# Autodesk Inventor assembly: Rail_AssemblyV2_0
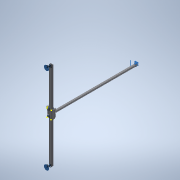
[picture p0: Inventor's stored thumbnail of the model, 180x180]
Saved by Autodesk Inventor 2021 (Build 250183000, 183)
## iProperties
Created: 2021-01-25
Part Number: Rail_AssemblyV2_0
Document SubType Name: Assembly
Designer: Jorian Brusind
Mass: 3786.54 g
Surface Area: 19508.5 cm^2
Volume: 2323.9 cm^3
Density: 1.62939 g/cm^3
Author: Jorian Brusind
## Documents named in this file (26)
- C:\Users\Jorian Bruslind\Documents\GitHub\PersonalProjects\HyperRail\Inventor Files\Rail_AssemblyV2_0.iam
- C:\Users\Jorian Bruslind\Documents\GitHub\PersonalProjects\Inventor Projects\Useful models\NEMA_Steppers\NEMA23\23HS8430B.ipt
- C:\Users\Jorian Bruslind\Documents\GitHub\PersonalProjects\HyperRail\Inventor Files\NEMA23_StepperonlineMount.ipt
- C:\Users\Jorian Bruslind\Documents\GitHub\PersonalProjects\Inventor Projects\Useful models\8020_Sets\IPT_20_Series\IPT_20_Series\20-2040_200mm.ipt
- C:\Users\Jorian Bruslind\Documents\GitHub\PersonalProjects\HyperRail\Inventor Files\2804S_NEMA2115_1Gearbox.ipt
- C:\Users\Jorian Bruslind\Documents\GitHub\PersonalProjects\HyperRail\Inventor Files\SmallBelt_LargePulley.ipt
- C:\Users\Jorian Bruslind\Documents\GitHub\PersonalProjects\HyperRail\PCB Files\Integrated Stepper Motor Driver\ExportSTEP\Main.iam
- C:\Users\Jorian Bruslind\Documents\GitHub\PersonalProjects\HyperRail\Inventor Files\NEMA23_Shroud.ipt
- C:\Users\Jorian Bruslind\Documents\GitHub\PersonalProjects\Inventor Projects\Useful models\8020_Sets\IPT_20_Series\IPT_20_Series\20-4040_2m.ipt
- C:\Users\Jorian Bruslind\Documents\GitHub\PersonalProjects\HyperRail\Inventor Files\98952A059_ALUM MALE-FEM THRDED HEX STANDOFF.ipt
- C:\Users\Jorian Bruslind\Documents\GitHub\PersonalProjects\HyperRail\Inventor Files\95783A039_NYLON 6-6 MALE-FEM THRDED HEX STANDOFF.ipt
- C:\Users\Jorian Bruslind\Documents\GitHub\PersonalProjects\HyperRail\Inventor Files\Integrated_Stepper_NEMA23_Mount.ipt
- C:\Users\Jorian Bruslind\Documents\GitHub\PersonalProjects\HyperRail\Inventor Files\Foot_Spacer.ipt
- C:\Users\Jorian Bruslind\Documents\GitHub\PersonalProjects\Inventor Projects\Useful models\Metric bolt\Bolt M5 50mm.ipt
- C:\Users\Jorian Bruslind\Documents\GitHub\PersonalProjects\Inventor Projects\Useful models\Metric nuts\Nut M5.ipt
- C:\Users\Jorian Bruslind\Documents\GitHub\PersonalProjects\HyperRail\Inventor Files\Bottom_Foot.ipt
- C:\Users\Jorian Bruslind\Documents\GitHub\PersonalProjects\HyperRail\Inventor Files\120deg_Tslot_Gusset.ipt
- C:\Users\Jorian Bruslind\Documents\GitHub\PersonalProjects\HyperRail\Inventor Files\90deg_4040Bracket.ipt
- C:\Users\Jorian Bruslind\Documents\GitHub\PersonalProjects\HyperRail\Inventor Files\X_Carriage_V2_0.iam
- C:\Users\Jorian Bruslind\Documents\GitHub\PersonalProjects\HyperRail\Inventor Files\11mm_BearingWheel.ipt
- C:\Users\Jorian Bruslind\Documents\GitHub\PersonalProjects\HyperRail\Inventor Files\X_CarriageR_V2_0.iam
- C:\Users\Jorian Bruslind\Documents\GitHub\PersonalProjects\Inventor Projects\Useful models\8020_Sets\IPT_40_Series\Extra_40_Series\HFS5-4060-4000\HFS5-4060-2125.ipt
- C:\Users\Jorian Bruslind\Documents\GitHub\PersonalProjects\Inventor Projects\Useful models\8020_Sets\IPT_20_Series\IPT_20_Series\20-2040_150mm.ipt
- C:\Users\Jorian Bruslind\Documents\GitHub\PersonalProjects\HyperRail\Inventor Files\RightAngle_Bracket_60mm.ipt
- C:\Users\Jorian Bruslind\Documents\GitHub\PersonalProjects\HyperRail\Inventor Files\X_CarriageR_V2_0_Short.iam
- C:\Users\Jorian Bruslind\Documents\GitHub\PersonalProjects\HyperRail\Inventor Files\X_CarriageL_V2_0_Short.iam
## Components (40 placed, 25 different names)
1. 23HS8430B:1 — Mate:127, Angle:3, Mate:158, Mate:177, Mate:179, Mate:180, Mate:181, Mate:182, Mate:183, Mate:184, Mate:185, Mate:264, Mate:265, Mate:295
2. NEMA23_StepperonlineMount:1 — Angle:2, Mate:98, Mate:128, Mate:255, Mate:258, Mate:259, Mate:289, Flush:99, Mate:290, Mate:303, Mate:304, Flush:107, Flush:108
3. 20-2040_200mm:1 — Mate:253, Flush:83, Flush:84, Flush:88, Mate:284, Mate:297, Mate:301, Mate:302, Flush:111, Flush:112
4. 2804S_NEMA2115_1Gearbox:1 — Angle:2, Mate:98, Mate:127, Mate:128, Angle:3, Mate:158, Mate:204, Flush:66, Flush:86
5. SmallBelt_LargePulley:1 — Mate:204, Flush:66
6. Main:1 [sub-assembly] — Mate:291, Mate:292, Mate:293
7. 20-4040_2m:2 — Mate:230, Flush:69, Flush:70, Mate:231, Flush:71, Flush:72, Mate:232, Flush:73, Mate:233, Mate:234, Flush:74, Mate:288, Flush:97, Flush:98
8. NEMA23_Shroud:1 — Mate:264, Mate:265, Flush:86, Mate:294
9. 98952A059_ALUM MALE-FEM THRDED HEX STANDOFF:1 — Mate:180, Mate:181, Mate:186, Mate:191
10. 98952A059_ALUM MALE-FEM THRDED HEX STANDOFF:2 — Mate:184, Mate:185, Mate:189, Mate:192
11. 98952A059_ALUM MALE-FEM THRDED HEX STANDOFF:3 — Mate:177, Mate:179, Mate:187, Mate:190
12. 98952A059_ALUM MALE-FEM THRDED HEX STANDOFF:4 — Mate:182, Mate:183, Mate:188, Mate:193
13. 95783A039_NYLON 6-6 MALE-FEM THRDED HEX STANDOFF:1 — Mate:188, Mate:193
14. 95783A039_NYLON 6-6 MALE-FEM THRDED HEX STANDOFF:2 — Mate:186, Mate:191
15. 95783A039_NYLON 6-6 MALE-FEM THRDED HEX STANDOFF:3 — Mate:187, Mate:190
16. 95783A039_NYLON 6-6 MALE-FEM THRDED HEX STANDOFF:4 — Mate:189, Mate:192
17. Bolt M5 50mm:1 — Mate:224, Mate:245, Mate:246, Mate:247, Mate:269
18. Nut M5:1 — Mate:226, Mate:247
19. Nut M5:2 — Mate:244, Flush:78, Mate:246
20. Bottom_Foot:1 — Mate:224, Mate:226, Mate:245, Flush:81, Flush:93
21. 120deg_Tslot_Gusset:1 — Mate:230, Flush:69, Flush:70
22. 120deg_Tslot_Gusset:2 — Mate:231, Flush:71, Flush:72
23. 90deg_4040Bracket:1 — Mate:232, Flush:73, Mate:233, Flush:75
24. 90deg_4040Bracket:2 — Mate:234, Flush:74, Flush:75
25. Foot_Spacer:1 — Mate:244, Flush:78, Mate:269, Mate:283, Flush:94
26. Foot_Spacer:2 — Mate:250, Mate:281, Flush:91, Flush:92, Mate:282
27. Bottom_Foot:2 — Mate:249, Mate:251, Flush:81, Flush:93
28. Bolt M5 50mm:2 — Mate:249, Mate:250, Mate:251, Mate:282
29. X_Carriage_V2_0:1 [sub-assembly] — Mate:253, Flush:83, Flush:84, Flush:109, Mate:309, Flush:113
30. 11mm_BearingWheel:1 — Mate:255, Mate:290
31. 11mm_BearingWheel:2 — Mate:258, Mate:259, Flush:109
32. 20-2040_200mm:2 — Flush:88, Mate:286, Flush:96, Mate:305, Flush:111, Mate:312, Flush:114
33. HFS5-4060-2125:1 — Mate:277, Mate:278, Mate:279, Mate:280, Mate:281, Flush:91, Flush:92, Mate:283, Flush:94, Mate:284, Flush:114
34. 20-2040_150mm:1 — Mate:286, Flush:96, Mate:288, Flush:97, Flush:98, Mate:289, Flush:99, Mate:310
35. Integrated_Stepper_NEMA23_Mount:1 — Mate:291, Mate:292, Mate:293, Mate:294, Mate:295
36. X_CarriageR_V2_0:2 [sub-assembly] — Mate:297, Mate:308, Flush:112, Flush:113, Mate:311
37. RightAngle_Bracket_60mm:1 — Mate:301, Mate:304, Flush:107
38. RightAngle_Bracket_60mm:2 — Mate:302, Mate:303, Flush:108
39. X_CarriageR_V2_0_Short:1 [sub-assembly] — Mate:305, Mate:308, Mate:309, Mate:310
40. X_CarriageL_V2_0_Short:1 [sub-assembly] — Mate:311, Mate:312
## Relationships (101: Mate 70, Flush 29, Angle 2)
- Angle:2 (0 deg): NEMA23_StepperonlineMount:1 ↔ 2804S_NEMA2115_1Gearbox:1
- Mate:98: NEMA23_StepperonlineMount:1 ↔ 2804S_NEMA2115_1Gearbox:1
- Mate:127: 23HS8430B:1 ↔ 2804S_NEMA2115_1Gearbox:1
- Mate:128: NEMA23_StepperonlineMount:1 ↔ 2804S_NEMA2115_1Gearbox:1
- Angle:3 (0 deg): 23HS8430B:1 ↔ 2804S_NEMA2115_1Gearbox:1
- Mate:158: 23HS8430B:1 ↔ 2804S_NEMA2115_1Gearbox:1
- Mate:177: 23HS8430B:1 ↔ 98952A059_ALUM MALE-FEM THRDED HEX STANDOFF:3
- Mate:179: 23HS8430B:1 ↔ 98952A059_ALUM MALE-FEM THRDED HEX STANDOFF:3
- Mate:180: 23HS8430B:1 ↔ 98952A059_ALUM MALE-FEM THRDED HEX STANDOFF:1
- Mate:181: 23HS8430B:1 ↔ 98952A059_ALUM MALE-FEM THRDED HEX STANDOFF:1
- Mate:182: 23HS8430B:1 ↔ 98952A059_ALUM MALE-FEM THRDED HEX STANDOFF:4
- Mate:183: 23HS8430B:1 ↔ 98952A059_ALUM MALE-FEM THRDED HEX STANDOFF:4
- Mate:184: 23HS8430B:1 ↔ 98952A059_ALUM MALE-FEM THRDED HEX STANDOFF:2
- Mate:185: 23HS8430B:1 ↔ 98952A059_ALUM MALE-FEM THRDED HEX STANDOFF:2
- Mate:186: 98952A059_ALUM MALE-FEM THRDED HEX STANDOFF:1 ↔ 95783A039_NYLON 6-6 MALE-FEM THRDED HEX STANDOFF:2
- Mate:187: 98952A059_ALUM MALE-FEM THRDED HEX STANDOFF:3 ↔ 95783A039_NYLON 6-6 MALE-FEM THRDED HEX STANDOFF:3
- Mate:188: 98952A059_ALUM MALE-FEM THRDED HEX STANDOFF:4 ↔ 95783A039_NYLON 6-6 MALE-FEM THRDED HEX STANDOFF:1
- Mate:189: 98952A059_ALUM MALE-FEM THRDED HEX STANDOFF:2 ↔ 95783A039_NYLON 6-6 MALE-FEM THRDED HEX STANDOFF:4
- Mate:190: 98952A059_ALUM MALE-FEM THRDED HEX STANDOFF:3 ↔ 95783A039_NYLON 6-6 MALE-FEM THRDED HEX STANDOFF:3
- Mate:191: 98952A059_ALUM MALE-FEM THRDED HEX STANDOFF:1 ↔ 95783A039_NYLON 6-6 MALE-FEM THRDED HEX STANDOFF:2
- Mate:192: 98952A059_ALUM MALE-FEM THRDED HEX STANDOFF:2 ↔ 95783A039_NYLON 6-6 MALE-FEM THRDED HEX STANDOFF:4
- Mate:193: 98952A059_ALUM MALE-FEM THRDED HEX STANDOFF:4 ↔ 95783A039_NYLON 6-6 MALE-FEM THRDED HEX STANDOFF:1
- Mate:204: 2804S_NEMA2115_1Gearbox:1 ↔ SmallBelt_LargePulley:1
- Flush:66: 2804S_NEMA2115_1Gearbox:1 ↔ SmallBelt_LargePulley:1
- Mate:224: Bolt M5 50mm:1 ↔ Bottom_Foot:1
- Mate:226: Nut M5:1 ↔ Bottom_Foot:1
- Mate:230: 20-4040_2m:2 ↔ 120deg_Tslot_Gusset:1
- Flush:69: 20-4040_2m:2 ↔ 120deg_Tslot_Gusset:1
- Flush:70: 20-4040_2m:2 ↔ 120deg_Tslot_Gusset:1
- Mate:231: 20-4040_2m:2 ↔ 120deg_Tslot_Gusset:2
- Flush:71: 20-4040_2m:2 ↔ 120deg_Tslot_Gusset:2
- Flush:72: 20-4040_2m:2 ↔ 120deg_Tslot_Gusset:2
- Mate:232: 20-4040_2m:2 ↔ 90deg_4040Bracket:1
- Flush:73: 20-4040_2m:2 ↔ 90deg_4040Bracket:1
- Mate:233: 20-4040_2m:2 ↔ 90deg_4040Bracket:1
- Mate:234: 20-4040_2m:2 ↔ 90deg_4040Bracket:2
- Flush:74: 20-4040_2m:2 ↔ 90deg_4040Bracket:2
- Flush:75: 90deg_4040Bracket:1 ↔ 90deg_4040Bracket:2
- Mate:244: Nut M5:2 ↔ Foot_Spacer:1
- Flush:78: Nut M5:2 ↔ Foot_Spacer:1
- Mate:245: Bolt M5 50mm:1 ↔ Bottom_Foot:1
- Mate:246: Bolt M5 50mm:1 ↔ Nut M5:2
- Mate:247: Bolt M5 50mm:1 ↔ Nut M5:1
- Mate:249: Bottom_Foot:2 ↔ Bolt M5 50mm:2
- Mate:250: Foot_Spacer:2 ↔ Bolt M5 50mm:2
- Mate:251: Bottom_Foot:2 ↔ Bolt M5 50mm:2
- Flush:81: Bottom_Foot:1 ↔ Bottom_Foot:2
- Mate:253: 20-2040_200mm:1 ↔ X_Carriage_V2_0:1
- Flush:83 (-30.5 mm): 20-2040_200mm:1 ↔ X_Carriage_V2_0:1
- Flush:84: 20-2040_200mm:1 ↔ X_Carriage_V2_0:1
- Mate:255 (13 mm): NEMA23_StepperonlineMount:1 ↔ 11mm_BearingWheel:1
- Mate:258: NEMA23_StepperonlineMount:1 ↔ 11mm_BearingWheel:2
- Mate:259 (13 mm): NEMA23_StepperonlineMount:1 ↔ 11mm_BearingWheel:2
- Mate:264 (1 mm): 23HS8430B:1 ↔ NEMA23_Shroud:1
- Mate:265 (1 mm): 23HS8430B:1 ↔ NEMA23_Shroud:1
- Mate:269: Bolt M5 50mm:1 ↔ Foot_Spacer:1
- Flush:86: 2804S_NEMA2115_1Gearbox:1 ↔ NEMA23_Shroud:1
- Flush:88: 20-2040_200mm:1 ↔ 20-2040_200mm:2
- Mate:277: HFS5-4060-2125:1
- Mate:278: HFS5-4060-2125:1
- Mate:279: HFS5-4060-2125:1
- Mate:280: HFS5-4060-2125:1
- Mate:281: Foot_Spacer:2 ↔ HFS5-4060-2125:1
- Flush:91: Foot_Spacer:2 ↔ HFS5-4060-2125:1
- Flush:92 (20 mm): Foot_Spacer:2 ↔ HFS5-4060-2125:1
- Mate:282: Foot_Spacer:2 ↔ Bolt M5 50mm:2
- Flush:93: Bottom_Foot:1 ↔ Bottom_Foot:2
- Mate:283 (-40 mm): Foot_Spacer:1 ↔ HFS5-4060-2125:1
- Flush:94: Foot_Spacer:1 ↔ HFS5-4060-2125:1
- Mate:284 (26 mm): 20-2040_200mm:1 ↔ HFS5-4060-2125:1
- Mate:286: 20-2040_200mm:2 ↔ 20-2040_150mm:1
- Flush:96: 20-2040_200mm:2 ↔ 20-2040_150mm:1
- Mate:288: 20-4040_2m:2 ↔ 20-2040_150mm:1
- Flush:97 (30 mm): 20-4040_2m:2 ↔ 20-2040_150mm:1
- Flush:98: 20-4040_2m:2 ↔ 20-2040_150mm:1
- Mate:289: NEMA23_StepperonlineMount:1 ↔ 20-2040_150mm:1
- Flush:99 (-12.5 mm): NEMA23_StepperonlineMount:1 ↔ 20-2040_150mm:1
- Mate:290: NEMA23_StepperonlineMount:1 ↔ 11mm_BearingWheel:1
- Mate:291: Main:1 ↔ Integrated_Stepper_NEMA23_Mount:1
- Mate:292: Main:1 ↔ Integrated_Stepper_NEMA23_Mount:1
- Mate:293: Main:1 ↔ Integrated_Stepper_NEMA23_Mount:1
- Mate:294: NEMA23_Shroud:1 ↔ Integrated_Stepper_NEMA23_Mount:1
- Mate:295: 23HS8430B:1 ↔ Integrated_Stepper_NEMA23_Mount:1
- Mate:297: 20-2040_200mm:1 ↔ X_CarriageR_V2_0:2
- Mate:301: 20-2040_200mm:1 ↔ RightAngle_Bracket_60mm:1
- Mate:302: 20-2040_200mm:1 ↔ RightAngle_Bracket_60mm:2
- Mate:303: NEMA23_StepperonlineMount:1 ↔ RightAngle_Bracket_60mm:2
- Mate:304: NEMA23_StepperonlineMount:1 ↔ RightAngle_Bracket_60mm:1
- Flush:107: NEMA23_StepperonlineMount:1 ↔ RightAngle_Bracket_60mm:1
- Flush:108: NEMA23_StepperonlineMount:1 ↔ RightAngle_Bracket_60mm:2
- Flush:109: X_Carriage_V2_0:1 ↔ 11mm_BearingWheel:2
- Mate:305: 20-2040_200mm:2 ↔ X_CarriageR_V2_0_Short:1
- Flush:111: 20-2040_200mm:1 ↔ 20-2040_200mm:2
- Mate:308 (25 mm): X_CarriageR_V2_0:2 ↔ X_CarriageR_V2_0_Short:1
- Mate:309: X_Carriage_V2_0:1 ↔ X_CarriageR_V2_0_Short:1
- Mate:310 (2.5 mm): 20-2040_150mm:1 ↔ X_CarriageR_V2_0_Short:1
- Flush:112: 20-2040_200mm:1 ↔ X_CarriageR_V2_0:2
- Flush:113: X_Carriage_V2_0:1 ↔ X_CarriageR_V2_0:2
- Mate:311: X_CarriageR_V2_0:2 ↔ X_CarriageL_V2_0_Short:1
- Mate:312: 20-2040_200mm:2 ↔ X_CarriageL_V2_0_Short:1
- Flush:114: 20-2040_200mm:2 ↔ HFS5-4060-2125:1
